# Autodesk Inventor assembly: fc17-151_Assembled
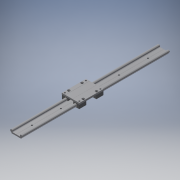
[picture p0: Inventor's stored thumbnail of the model, 180x180]
Saved by Autodesk Inventor 2017.1 (Build 211199000, 199)
## iProperties
Category: Miscellaneous
Company: Autodesk Inc.
Created: 2016-12-21
Part Number: fc17-151_Assembled
Document SubType Name: Assembly
Designer: Autodesk Inc.
Catalog Web Link: http://www.igus.com/wpck/3624/DryLin_W_Doppelschiene
Vendor: AndyMark Inc.
Author: Autodesk Inc.
Keywords: FIRST Choice
## Documents named in this file (3)
- D:\FIRST\FIRST KOP 2017\FIRST FirstChoice 2017\fc17-151_Assembled.iam
- D:\FIRST\FIRST KOP 2017\FIRST FirstChoice 2017\fc17-151_Rail.ipt
- D:\FIRST\FIRST KOP 2017\FIRST FirstChoice 2017\fc17-151_Carriage.ipt
## Components (2 placed, 2 different names)
1. fc17-151_Rail:1 — Mate:1, Mate:2
2. fc17-151_Carriage:1 — Mate:1, Mate:2
## Relationships (2: Mate 2)
- Mate:1: fc17-151_Rail:1 ↔ fc17-151_Carriage:1
- Mate:2: fc17-151_Rail:1 ↔ fc17-151_Carriage:1
